# Autodesk Inventor assembly: Lift.03.01.01.00
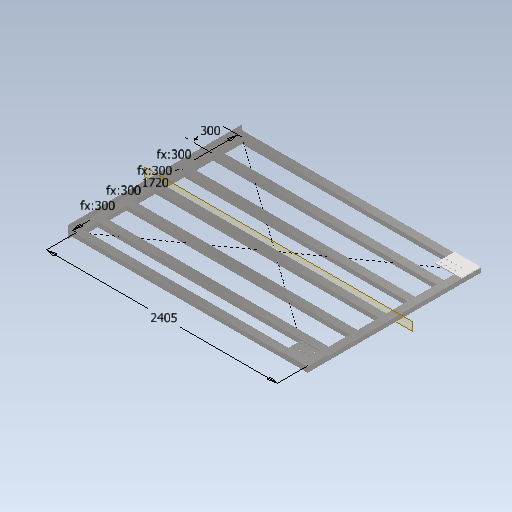
[picture p0: Inventor's stored thumbnail of the model, 512x512]
Saved by Autodesk Inventor 2021 (Build 250183000, 183)
## iProperties
Created: 2020-09-20
Part Number: Lift.03.01.01.00
Document SubType Name: Assembly
Designer: Kostya
_SolveAssemblyDoc: Frame Generator Solve Assembly
_Version: 25.0.0
Author: Kostya
## Documents named in this file (6)
- C:\Lift\Lift.03.01.01.00.iam
- C:\Lift\Lift.03.01.00.02.ipt
- C:\Lift\Lift.03.01.01.01.ipt
- C:\Lift\Lift.03.01.00.03.ipt
- C:\Lift\Lift.03.01.00.02_MIR.ipt
- C:\Lift\Lift.03.01.01.00\Frame\Frame 1600622446614.iam
## Components (5 placed, 5 different names)
1. Lift.03.01.00.02:1 — Заподлицо:3, Заподлицо:4, Совмещение:3
2. Lift.03.01.01.01:1
3. Lift.03.01.00.03:1 — Заподлицо:1, Совмещение:1, Заподлицо:2
4. Lift.03.01.00.02_MIR:1 — Заподлицо:5, Заподлицо:6, Совмещение:2
5. Frame 1600622446614:1 [sub-assembly] — Заподлицо:1, Совмещение:1, Заподлицо:2, Заподлицо:3, Заподлицо:4, Заподлицо:5, Заподлицо:6, Совмещение:2, Совмещение:3
## Relationships (9: Flush 6, Mate 3)
- Заподлицо:1 [Flush]: Lift.03.01.00.03:1 ↔ Frame 1600622446614:1
- Совмещение:1 [Mate]: Lift.03.01.00.03:1 ↔ Frame 1600622446614:1
- Заподлицо:2 [Flush] (40 mm): Lift.03.01.00.03:1 ↔ Frame 1600622446614:1
- Заподлицо:3 [Flush]: Lift.03.01.00.02:1 ↔ Frame 1600622446614:1
- Заподлицо:4 [Flush]: Lift.03.01.00.02:1 ↔ Frame 1600622446614:1
- Заподлицо:5 [Flush]: Lift.03.01.00.02_MIR:1 ↔ Frame 1600622446614:1
- Заподлицо:6 [Flush]: Lift.03.01.00.02_MIR:1 ↔ Frame 1600622446614:1
- Совмещение:2 [Mate]: Lift.03.01.00.02_MIR:1 ↔ Frame 1600622446614:1
- Совмещение:3 [Mate]: Lift.03.01.00.02:1 ↔ Frame 1600622446614:1
